# Autodesk Inventor assembly: model tensometru
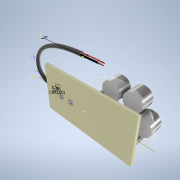
[picture p0: Inventor's stored thumbnail of the model, 180x180]
Saved by Autodesk Inventor 2021 (Build 250183000, 183)
## iProperties
Created: 2021-11-16
Part Number: model tensometru
Document SubType Name: Assembly
Designer: wojwo
Author: wojwo
## Documents named in this file (9)
- D:\OneDrive\Studia\5 semestr\ARMIKO\lab2\model3d\model tensometru.iam
- D:\OneDrive\Studia\5 semestr\ARMIKO\lab2\model3d\tensometr.ipt
- D:\OneDrive\Studia\5 semestr\ARMIKO\lab2\model3d\podstwa.ipt
- D:\OneDrive\Studia\5 semestr\ARMIKO\lab2\model3d\szklo.ipt
- D:\Dokumenty\Inventor\Content Center Files\R2021\pl-PL\ISO 10642(1)\ISO 10642 - M4x12.ipt
- D:\OneDrive\Studia\5 semestr\ARMIKO\lab2\model3d\zalany_tensometr.ipt
- D:\OneDrive\Studia\5 semestr\ARMIKO\lab2\model3d\kabelki.ipt
- D:\OneDrive\Studia\5 semestr\ARMIKO\lab2\model3d\kabel.ipt
- D:\OneDrive\Studia\5 semestr\ARMIKO\lab2\model3d\ciezarek.ipt
## Components (16 placed, 8 different names)
1. tensometr:1 — Równoległe:2, Równoległe:3, Równoległe:6, Równoległe:7, Zestawiające:6
2. podstwa:1 — Równoległe:1, Zestawiające:1, Zestawiające:2, Zestawiające:3, Równoległe:5, Równoległe:21, Równoległe:22, Równoległe:23, Równoległe:24, Równoległe:25
3. szklo:1 — Równoległe:2, Równoległe:3, Zestawiające:4, Zestawiające:5, Równoległe:26
4. ISO 10642 M4x12:1 — Zestawiające:1, Równoległe:4, Zestawiające:3, Równoległe:5
5. ISO 10642 M4x12:2 — Zestawiające:2, Równoległe:4
6. ISO 10642 M4x12:3 — Zestawiające:4
7. ISO 10642 M4x12:4 — Zestawiające:5
8. zalany_tensometr:1 — Równoległe:6, Równoległe:7, Równoległe:8, Równoległe:9, Równoległe:10, Równoległe:11, Równoległe:12, Równoległe:13
9. kabelki:1 — Równoległe:8, Równoległe:9, Równoległe:10, Równoległe:11, Równoległe:12, Równoległe:13, Równoległe:15, Równoległe:16, Zestawiające:6, Zestawiające:7, Zestawiające:8
10. kabel:1 — Równoległe:17, Równoległe:18, Zestawiające:7, Zestawiające:8, Zestawiające:9, Kątowe:1, Równoległe:20, Równoległe:21, Równoległe:22, Równoległe:23, Równoległe:24, Równoległe:25
11. ciezarek:1 — Równoległe:26
12. ciezarek:2
13. ciezarek:3
14. ciezarek:4
15. ciezarek:5
16. ciezarek:6
## Component patterns: (6 elements, first: ciezarek:1)
## Relationships (35: Flush 25, Mate 9, Angle 1)
- Równoległe:1 [Flush]: podstwa:1
- Równoległe:2 [Flush]: tensometr:1 ↔ szklo:1
- Równoległe:3 [Flush]: tensometr:1 ↔ szklo:1
- Zestawiające:1 [Mate]: podstwa:1 ↔ ISO 10642 M4x12:1
- Zestawiające:2 [Mate]: podstwa:1 ↔ ISO 10642 M4x12:2
- Równoległe:4 [Flush]: ISO 10642 M4x12:1 ↔ ISO 10642 M4x12:2
- Zestawiające:3 [Mate]: podstwa:1 ↔ ISO 10642 M4x12:1
- Równoległe:5 [Flush]: podstwa:1 ↔ ISO 10642 M4x12:1
- Zestawiające:4 [Mate]: szklo:1 ↔ ISO 10642 M4x12:3
- Zestawiające:5 [Mate]: szklo:1 ↔ ISO 10642 M4x12:4
- Równoległe:6 [Flush]: tensometr:1 ↔ zalany_tensometr:1
- Równoległe:7 [Flush]: tensometr:1 ↔ zalany_tensometr:1
- Równoległe:8 [Flush]: zalany_tensometr:1 ↔ kabelki:1
- Równoległe:9 [Flush] (20 mm): zalany_tensometr:1 ↔ kabelki:1
- Równoległe:10 [Flush]: zalany_tensometr:1 ↔ kabelki:1
- Równoległe:11 [Flush]: zalany_tensometr:1 ↔ kabelki:1
- Równoległe:12 [Flush]: zalany_tensometr:1 ↔ kabelki:1
- Równoległe:13 [Flush]: zalany_tensometr:1 ↔ kabelki:1
- Równoległe:14 [Flush] (-5 mm)
- Równoległe:15 [Flush]: kabelki:1
- Równoległe:16 [Flush]: kabelki:1
- Zestawiające:6 [Mate]: tensometr:1 ↔ kabelki:1
- Równoległe:17 [Flush]: kabel:1
- Równoległe:18 [Flush]: kabel:1
- Zestawiające:7 [Mate]: kabelki:1 ↔ kabel:1
- Zestawiające:8 [Mate]: kabelki:1 ↔ kabel:1
- Zestawiające:9 [Mate]: kabel:1
- Kątowe:1 [Angle] (90 deg): kabel:1
- Równoległe:20 [Flush]: kabel:1
- Równoległe:21 [Flush]: podstwa:1 ↔ kabel:1
- Równoległe:22 [Flush] (30 mm): podstwa:1 ↔ kabel:1
- Równoległe:23 [Flush] (30 mm): podstwa:1 ↔ kabel:1
- Równoległe:24 [Flush]: podstwa:1 ↔ kabel:1
- Równoległe:25 [Flush]: podstwa:1 ↔ kabel:1
- Równoległe:26 [Flush]: szklo:1 ↔ ciezarek:1
